# Autodesk Inventor assembly: RC Assembly
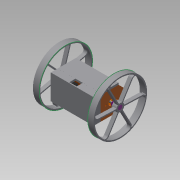
[picture p0: Inventor's stored thumbnail of the model, 180x180]
Saved by Autodesk Inventor 2019.3 (Build 233278000, 278)
## iProperties
Created: 2019-05-20
Part Number: RC Assembly
Document SubType Name: Assembly
Designer: Johansson
Author: Johansson
## Documents named in this file (5)
- C:\Users\oskar\Dropbox\Dokument\Projekt\RC Two Wheeler\RC-two-wheeler\CAD\RC Assembly.iam
- C:\Users\oskar\Dropbox\Dokument\Projekt\RC Two Wheeler\RC-two-wheeler\CAD\KEDA_6364.ipt
- C:\Users\oskar\Dropbox\Dokument\Projekt\RC Two Wheeler\RC-two-wheeler\CAD\Platform.ipt
- C:\Users\oskar\Dropbox\Dokument\Projekt\RC Two Wheeler\RC-two-wheeler\CAD\Wheel.ipt
- C:\Users\oskar\Dropbox\Dokument\Projekt\RC Two Wheeler\RC-two-wheeler\CAD\NESE 2S2P.ipt
## Components (7 placed, 4 different names)
1. KEDA_6364:1 — Mate:1, Mate:2, Mate:3, Mate:7
2. Platform:1 — Mate:1, Mate:2, Mate:3, Mate:4, Mate:5, Mate:6, Mate:9, Mate:10, Mate:11, Mate:12
3. KEDA_6364:2 — Mate:4, Mate:5, Mate:6, Mate:8
4. Wheel:1 — Mate:7
5. Wheel:2 — Mate:8
6. NESE 2S2P:1 — Mate:11, Mate:12
7. NESE 2S2P:2 — Mate:9, Mate:10
## Relationships (12: Mate 12)
- Mate:1: KEDA_6364:1 ↔ Platform:1
- Mate:2: KEDA_6364:1 ↔ Platform:1
- Mate:3: KEDA_6364:1 ↔ Platform:1
- Mate:4: Platform:1 ↔ KEDA_6364:2
- Mate:5: Platform:1 ↔ KEDA_6364:2
- Mate:6: Platform:1 ↔ KEDA_6364:2
- Mate:7 (-10 mm): KEDA_6364:1 ↔ Wheel:1
- Mate:8 (-10 mm): KEDA_6364:2 ↔ Wheel:2
- Mate:9: Platform:1 ↔ NESE 2S2P:2
- Mate:10: Platform:1 ↔ NESE 2S2P:2
- Mate:11: Platform:1 ↔ NESE 2S2P:1
- Mate:12: Platform:1 ↔ NESE 2S2P:1
